# Autodesk Inventor assembly: FEIBOT
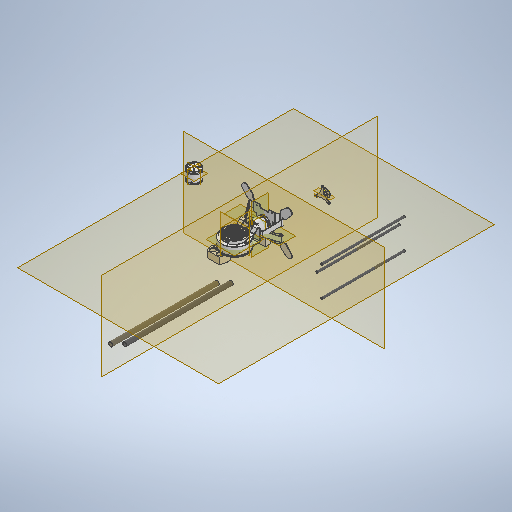
[picture p0: Inventor's stored thumbnail of the model, 512x512]
Saved by Autodesk Inventor 2025.3 (Build 293356000, 356)
## iProperties
Created: 2026-08-06
Part Number: FEIBOT
Document SubType Name: Assembly
Designer: Admin
Author: Admin
## Documents named in this file (12)
- C:\Users\shfzf\Desktop\FEIBOT\ROBOT_CAD\FEIBOT.iam
- C:\Users\shfzf\Desktop\FEIBOT\ROBOT_CAD\BASE\BASE.ipt
- C:\Users\shfzf\Desktop\FEIBOT\ROBOT_CAD\DM-J4340\DM-J4340.iam
- C:\Users\shfzf\Desktop\FEIBOT\ROBOT_CAD\DM-J10010l\DM-J10010l.iam
- C:\Users\shfzf\Desktop\FEIBOT\ROBOT_CAD\J1_J2_FLANGE\J1_J2_FLANGE.ipt
- C:\Users\shfzf\Desktop\FEIBOT\ROBOT_CAD\CARBON_TUBE\CARBON_TUBE_20MM.ipt
- C:\Users\shfzf\Desktop\FEIBOT\ROBOT_CAD\DC_DC_POWER.ipt
- C:\Users\shfzf\Desktop\FEIBOT\ROBOT_CAD\CARBON_TUBE\CARBON_TUBE.ipt
- C:\Users\shfzf\Desktop\FEIBOT\ROBOT_CAD\J4_CAR_CONNECTOR\J4_CAR_CONNECTOR.ipt
- C:\Users\shfzf\Desktop\FEIBOT\ROBOT_CAD\J1_J2_GASKET\J1_J2_GASKET.ipt
- C:\Users\shfzf\Desktop\FEIBOT\ROBOT_CAD\J2_HOLDER\J2_HOLDER.ipt
- C:\Users\shfzf\Desktop\FEIBOT\ROBOT_CAD\J2_CAR_CONNECTOR\J2_CAR_CONNECTOR.ipt
## Components (15 placed, 11 different names)
1. BASE:1 — 配合:1, 配合:2, 配合:3, 配合:4, 配合:5, 配合:6, 配合:22, 配合:23, 配合:24
2. DM-J4340:1 [sub-assembly]
3. DM-J4340:2 [sub-assembly] — 配合:4, 配合:5, 配合:6, 配合:7, 配合:8, 配合:35
4. DM-J10010l:1 [sub-assembly] — 配合:31, 配合:32, 配合:33, 配合:34
5. J1_J2_FLANGE:1 — 配合:7, 配合:8, 配合:25, 配合:26, 配合:30
6. DC_DC_POWER:1 — 配合:22, 配合:23, 配合:24
7. J4_CAR_CONNECTOR:1
8. J1_J2_GASKET:1 — 配合:25, 配合:26, 配合:27, 配合:28, 配合:29, 配合:35
9. J2_HOLDER:1 — 配合:27, 配合:28, 配合:29, 配合:30, 配合:31, 配合:32, 配合:33, 配合:34
10. J2_CAR_CONNECTOR:1
11. CARBON_TUBE_20MM:1
12. CARBON_TUBE_20MM:2
13. CARBON_TUBE:1
14. CARBON_TUBE:2
15. CARBON_TUBE:3
## Relationships (22: Mate 22)
- 配合:1 [Mate]: BASE:1
- 配合:2 [Mate]: BASE:1
- 配合:3 [Mate]: BASE:1
- 配合:4 [Mate]: BASE:1 ↔ DM-J4340:2
- 配合:5 [Mate]: BASE:1 ↔ DM-J4340:2
- 配合:6 [Mate]: BASE:1 ↔ DM-J4340:2
- 配合:7 [Mate]: DM-J4340:2 ↔ J1_J2_FLANGE:1
- 配合:8 [Mate]: DM-J4340:2 ↔ J1_J2_FLANGE:1
- 配合:22 [Mate]: BASE:1 ↔ DC_DC_POWER:1
- 配合:23 [Mate]: BASE:1 ↔ DC_DC_POWER:1
- 配合:24 [Mate]: BASE:1 ↔ DC_DC_POWER:1
- 配合:25 [Mate]: J1_J2_FLANGE:1 ↔ J1_J2_GASKET:1
- 配合:26 [Mate]: J1_J2_FLANGE:1 ↔ J1_J2_GASKET:1
- 配合:27 [Mate]: J1_J2_GASKET:1 ↔ J2_HOLDER:1
- 配合:28 [Mate]: J1_J2_GASKET:1 ↔ J2_HOLDER:1
- 配合:29 [Mate]: J1_J2_GASKET:1 ↔ J2_HOLDER:1
- 配合:30 [Mate]: J1_J2_FLANGE:1 ↔ J2_HOLDER:1
- 配合:31 [Mate]: DM-J10010l:1 ↔ J2_HOLDER:1
- 配合:32 [Mate]: DM-J10010l:1 ↔ J2_HOLDER:1
- 配合:33 [Mate]: DM-J10010l:1 ↔ J2_HOLDER:1
- 配合:34 [Mate]: DM-J10010l:1 ↔ J2_HOLDER:1
- 配合:35 [Mate]: DM-J4340:2 ↔ J1_J2_GASKET:1
